# Autodesk Inventor assembly: fullcase
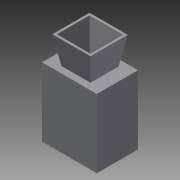
[picture p0: Inventor's stored thumbnail of the model, 180x180]
Saved by Autodesk Inventor 2017 (Build 210142000, 142)
## iProperties
Created: 2017-01-02
Part Number: fullcase
Document SubType Name: Assembly
Designer: Sachin Konan
Author: Sachin Konan
## Documents named in this file (3)
- C:\Users\Sachin Konan\Documents\ScienceFair2017\CADFIles\fullcase.iam
- C:\Users\Sachin Konan\Documents\ScienceFair2017\CADFIles\Antenna.ipt
- C:\Users\Sachin Konan\Documents\ScienceFair2017\CADFIles\case.ipt
## Components (2 placed, 2 different names)
1. Antenna:1 — Mate:1, Mate:2, Mate:3
2. case:1 — Mate:1, Mate:2, Mate:3
## Relationships (3: Mate 3)
- Mate:1: Antenna:1 ↔ case:1
- Mate:2: Antenna:1 ↔ case:1
- Mate:3: Antenna:1 ↔ case:1
